# Autodesk Inventor assembly: pcb_assembled
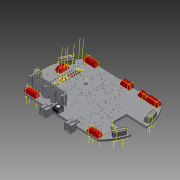
[picture p0: Inventor's stored thumbnail of the model, 180x180]
Saved by Autodesk Inventor 2014 (Build 180170000, 170)
## iProperties
Created: 2013-08-24
Part Number: pcb_assembled
Document SubType Name: Assembly
Designer: Felix
Author: Felix
## Documents named in this file (12)
- C:\Users\hanse\Desktop\Beep\Hardware\3D-CAD\parts\electronic\BEEP\beep_main_assembled.iam
- C:\Users\hanse\Desktop\Beep\Hardware\3D-CAD\parts\electronic\BEEP\components\8526-4500pl-01.ipt
- C:\Users\hanse\Desktop\Beep\Hardware\3D-CAD\parts\electronic\BEEP\components\micro-miniature_steckverbinder_a-32-08v-130x0.ipt
- C:\Users\hanse\Desktop\Beep\Hardware\3D-CAD\parts\electronic\BEEP\components\c-215460-8-h-3d.ipt
- C:\Users\hanse\Desktop\Beep\Hardware\3D-CAD\parts\electronic\BEEP\components\micro-miniature_steckverbinder_a-32-04v-130x0.ipt
- C:\Users\hanse\Desktop\Beep\Hardware\3D-CAD\parts\electronic\BEEP\components\micro-miniature_steckverbinder_a-32-06v-130x0.ipt
- C:\Users\hanse\Desktop\Beep\Hardware\3D-CAD\parts\electronic\BEEP\components\micro-miniature_steckverbinder_a-32-10v-130x0.ipt
- C:\Users\hanse\Desktop\Beep\Hardware\3D-CAD\parts\electronic\BEEP\components\12520.ipt
- C:\Users\hanse\Desktop\Beep\Hardware\3D-CAD\parts\electronic\BEEP\components\12521.ipt
- C:\Users\hanse\Desktop\Beep\Hardware\3D-CAD\parts\electronic\BEEP\components\b3w-1000.ipt
- C:\Users\hanse\Desktop\Beep\Hardware\3D-CAD\parts\electronic\BEEP\beep_main_new.ipt
- C:\Users\hanse\Desktop\Beep\Hardware\3D-CAD\parts\electronic\BEEP\components\cny-70.ipt
## Components (20 placed, 11 different names)
1. 8526-4500pl-01:1 — Passend:188, Passend:189, Passend:190
2. micro-miniature_steckverbinder_a-32-08v-130x0:1 — Passend:112, Passend:113, Passend:114, Passend:115
3. micro-miniature_steckverbinder_a-32-08v-130x0:2 — Passend:116, Passend:117, Passend:118, Passend:119
4. micro-miniature_steckverbinder_a-32-08v-130x0:3 — Passend:120, Passend:121, Passend:122, Passend:123
5. micro-miniature_steckverbinder_a-32-08v-130x0:4 — Passend:132, Passend:133, Passend:134, Passend:135
6. c-215460-8-h-3d:1 — Passend:149, Passend:151, Passend:152, Passend:153
7. c-215460-8-h-3d:2 — Passend:141, Passend:142, Passend:143, Passend:144
8. c-215460-8-h-3d:3 — Passend:146, Passend:147, Passend:148, Passend:158
9. c-215460-8-h-3d:4 — Passend:150, Passend:154, Passend:155, Passend:156, Passend:157
10. micro-miniature_steckverbinder_a-32-04v-130x0:1 — Passend:124, Passend:125, Passend:126, Passend:127
11. micro-miniature_steckverbinder_a-32-04v-130x0:2 — Passend:182, Passend:183, Passend:184, Passend:185
12. micro-miniature_steckverbinder_a-32-06v-130x0:1 — Passend:128, Passend:129, Passend:130, Passend:131
13. micro-miniature_steckverbinder_a-32-10v-130x0:1 — Passend:175, Passend:176, Passend:177, Passend:178
14. 12520:1 — Passend:163, Passend:164, Passend:165
15. 12521:1 — Passend:166, Passend:167, Passend:168
16. micro-miniature_steckverbinder_a-32-06v-130x0:2 — Passend:136, Passend:137, Passend:139, Passend:140
17. b3w-1000:1 — Passend:191
18. beep_main_new:1 — Passend:112, Passend:113, Passend:114, Passend:115, Passend:116, Passend:117, Passend:118, Passend:119, Passend:120, Passend:121, Passend:122, Passend:123, Passend:124, Passend:125, Passend:126, Passend:127, Passend:128, Passend:129, Passend:130, Passend:131, Passend:132, Passend:133, Passend:134, Passend:135, Passend:136, Passend:137, Passend:139, Passend:140, Passend:141, Passend:142, Passend:143, Passend:144, Passend:146, Passend:147, Passend:148, Passend:149, Passend:150, Passend:151, Passend:152, Passend:153, Passend:154, Passend:155, Passend:156, Passend:157, Passend:158, Passend:159, Passend:160, Passend:161, Passend:162, Passend:164, Passend:166, Passend:169, Passend:170, Passend:171, Passend:172, Passend:173, Passend:174, Passend:178, Passend:179, Passend:180, Passend:181, Passend:185, Passend:186, Passend:187, Passend:188, Passend:191, Passend:192, Passend:193, Passend:194, Passend:195, Passend:196, Passend:197
19. cny-70:1 — Passend:195, Passend:196
20. cny-70:2 — Passend:194, Passend:197
## Relationships (84: Mate 84)
- Passend:112 [Mate]: micro-miniature_steckverbinder_a-32-08v-130x0:1 ↔ beep_main_new:1
- Passend:113 [Mate]: micro-miniature_steckverbinder_a-32-08v-130x0:1 ↔ beep_main_new:1
- Passend:114 [Mate]: micro-miniature_steckverbinder_a-32-08v-130x0:1 ↔ beep_main_new:1
- Passend:115 [Mate]: micro-miniature_steckverbinder_a-32-08v-130x0:1 ↔ beep_main_new:1
- Passend:116 [Mate]: micro-miniature_steckverbinder_a-32-08v-130x0:2 ↔ beep_main_new:1
- Passend:117 [Mate]: micro-miniature_steckverbinder_a-32-08v-130x0:2 ↔ beep_main_new:1
- Passend:118 [Mate]: micro-miniature_steckverbinder_a-32-08v-130x0:2 ↔ beep_main_new:1
- Passend:119 [Mate]: micro-miniature_steckverbinder_a-32-08v-130x0:2 ↔ beep_main_new:1
- Passend:120 [Mate]: micro-miniature_steckverbinder_a-32-08v-130x0:3 ↔ beep_main_new:1
- Passend:121 [Mate]: micro-miniature_steckverbinder_a-32-08v-130x0:3 ↔ beep_main_new:1
- Passend:122 [Mate]: micro-miniature_steckverbinder_a-32-08v-130x0:3 ↔ beep_main_new:1
- Passend:123 [Mate]: micro-miniature_steckverbinder_a-32-08v-130x0:3 ↔ beep_main_new:1
- Passend:124 [Mate]: micro-miniature_steckverbinder_a-32-04v-130x0:1 ↔ beep_main_new:1
- Passend:125 [Mate]: micro-miniature_steckverbinder_a-32-04v-130x0:1 ↔ beep_main_new:1
- Passend:126 [Mate]: micro-miniature_steckverbinder_a-32-04v-130x0:1 ↔ beep_main_new:1
- Passend:127 [Mate]: micro-miniature_steckverbinder_a-32-04v-130x0:1 ↔ beep_main_new:1
- Passend:128 [Mate]: micro-miniature_steckverbinder_a-32-06v-130x0:1 ↔ beep_main_new:1
- Passend:129 [Mate]: micro-miniature_steckverbinder_a-32-06v-130x0:1 ↔ beep_main_new:1
- Passend:130 [Mate]: micro-miniature_steckverbinder_a-32-06v-130x0:1 ↔ beep_main_new:1
- Passend:131 [Mate]: micro-miniature_steckverbinder_a-32-06v-130x0:1 ↔ beep_main_new:1
- Passend:132 [Mate]: micro-miniature_steckverbinder_a-32-08v-130x0:4 ↔ beep_main_new:1
- Passend:133 [Mate]: micro-miniature_steckverbinder_a-32-08v-130x0:4 ↔ beep_main_new:1
- Passend:134 [Mate]: micro-miniature_steckverbinder_a-32-08v-130x0:4 ↔ beep_main_new:1
- Passend:135 [Mate]: micro-miniature_steckverbinder_a-32-08v-130x0:4 ↔ beep_main_new:1
- Passend:136 [Mate]: micro-miniature_steckverbinder_a-32-06v-130x0:2 ↔ beep_main_new:1
- Passend:137 [Mate]: micro-miniature_steckverbinder_a-32-06v-130x0:2 ↔ beep_main_new:1
- Passend:139 [Mate]: micro-miniature_steckverbinder_a-32-06v-130x0:2 ↔ beep_main_new:1
- Passend:140 [Mate]: micro-miniature_steckverbinder_a-32-06v-130x0:2 ↔ beep_main_new:1
- Passend:141 [Mate]: c-215460-8-h-3d:2 ↔ beep_main_new:1
- Passend:142 [Mate]: c-215460-8-h-3d:2 ↔ beep_main_new:1
- Passend:143 [Mate]: c-215460-8-h-3d:2 ↔ beep_main_new:1
- Passend:144 [Mate]: c-215460-8-h-3d:2 ↔ beep_main_new:1
- Passend:146 [Mate]: c-215460-8-h-3d:3 ↔ beep_main_new:1
- Passend:147 [Mate]: c-215460-8-h-3d:3 ↔ beep_main_new:1
- Passend:148 [Mate]: c-215460-8-h-3d:3 ↔ beep_main_new:1
- Passend:149 [Mate]: c-215460-8-h-3d:1 ↔ beep_main_new:1
- Passend:150 [Mate]: c-215460-8-h-3d:4 ↔ beep_main_new:1
- Passend:151 [Mate]: c-215460-8-h-3d:1 ↔ beep_main_new:1
- Passend:152 [Mate]: c-215460-8-h-3d:1 ↔ beep_main_new:1
- Passend:153 [Mate]: c-215460-8-h-3d:1 ↔ beep_main_new:1
- Passend:154 [Mate]: c-215460-8-h-3d:4 ↔ beep_main_new:1
- Passend:155 [Mate]: c-215460-8-h-3d:4 ↔ beep_main_new:1
- Passend:156 [Mate]: c-215460-8-h-3d:4 ↔ beep_main_new:1
- Passend:157 [Mate]: c-215460-8-h-3d:4 ↔ beep_main_new:1
- Passend:158 [Mate]: c-215460-8-h-3d:3 ↔ beep_main_new:1
- Passend:159 [Mate]: beep_main_new:1
- Passend:160 [Mate]: beep_main_new:1
- Passend:161 [Mate]: beep_main_new:1
- Passend:162 [Mate]: beep_main_new:1
- Passend:163 [Mate]: 12520:1
- Passend:164 [Mate]: 12520:1 ↔ beep_main_new:1
- Passend:165 [Mate]: 12520:1
- Passend:166 [Mate]: 12521:1 ↔ beep_main_new:1
- Passend:167 [Mate]: 12521:1
- Passend:168 [Mate]: 12521:1
- Passend:169 [Mate]: beep_main_new:1
- Passend:170 [Mate]: beep_main_new:1
- Passend:171 [Mate]: beep_main_new:1
- Passend:172 [Mate]: beep_main_new:1
- Passend:173 [Mate]: beep_main_new:1
- Passend:174 [Mate]: beep_main_new:1
- Passend:175 [Mate]: micro-miniature_steckverbinder_a-32-10v-130x0:1
- Passend:176 [Mate]: micro-miniature_steckverbinder_a-32-10v-130x0:1
- Passend:177 [Mate]: micro-miniature_steckverbinder_a-32-10v-130x0:1
- Passend:178 [Mate]: micro-miniature_steckverbinder_a-32-10v-130x0:1 ↔ beep_main_new:1
- Passend:179 [Mate]: beep_main_new:1
- Passend:180 [Mate]: beep_main_new:1
- Passend:181 [Mate]: beep_main_new:1
- Passend:182 [Mate]: micro-miniature_steckverbinder_a-32-04v-130x0:2
- Passend:183 [Mate]: micro-miniature_steckverbinder_a-32-04v-130x0:2
- Passend:184 [Mate]: micro-miniature_steckverbinder_a-32-04v-130x0:2
- Passend:185 [Mate]: micro-miniature_steckverbinder_a-32-04v-130x0:2 ↔ beep_main_new:1
- Passend:186 [Mate]: beep_main_new:1
- Passend:187 [Mate]: beep_main_new:1
- Passend:188 [Mate]: 8526-4500pl-01:1 ↔ beep_main_new:1
- Passend:189 [Mate]: 8526-4500pl-01:1
- Passend:190 [Mate]: 8526-4500pl-01:1
- Passend:191 [Mate]: b3w-1000:1 ↔ beep_main_new:1
- Passend:192 [Mate]: beep_main_new:1
- Passend:193 [Mate]: beep_main_new:1
- Passend:194 [Mate]: beep_main_new:1 ↔ cny-70:2
- Passend:195 [Mate]: beep_main_new:1 ↔ cny-70:1
- Passend:196 [Mate]: beep_main_new:1 ↔ cny-70:1
- Passend:197 [Mate]: beep_main_new:1 ↔ cny-70:2
